# Autodesk Inventor assembly: battery
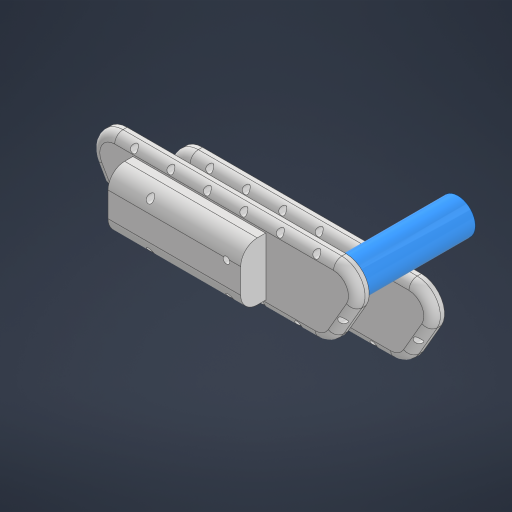
[picture p0: Inventor's stored thumbnail of the model, 512x512]
Saved by Autodesk Inventor 2024 (Build 280153000, 153)
## iProperties
Created: 2024-05-04
Part Number: battery
Document SubType Name: Assembly
Designer: markm
Author: markm
## Documents named in this file (6)
- C:\Users\markm\OneDrive\Документы\Inventor\eventide\back\battery\battery.iam
- C:\Users\markm\OneDrive\Документы\Inventor\eventide\back\battery\cell.ipt
- C:\Users\markm\OneDrive\Документы\Inventor\eventide\back\battery\frame.ipt
- C:\Users\markm\OneDrive\Документы\Inventor\eventide\back\battery\box.ipt
- C:\Users\markm\OneDrive\Документы\Inventor\eventide\back\battery\Part2.ipt
- C:\Users\markm\OneDrive\Документы\Inventor\eventide\back\battery\Part3.ipt
## Components (17 placed, 5 different names)
1. frame:1 — Mate:1, Mate:2, Flush:4, Flush:5, Mate:3, Mate:4, Mate:5
2. cell:2 — Mate:2, Flush:5
3. box:1 — Mate:3, Mate:4, Mate:5
4. Part2:1
5. Part3:1
6. cell:1 — Mate:1, Flush:4
7. cell:3
8. cell:4
9. cell:5
10. cell:6
11. cell:7
12. cell:8
13. cell:9
14. cell:10
15. cell:11
16. cell:12
17. cell:13
## Component patterns: (12 elements, first: cell:1)
## Relationships (7: Mate 5, Flush 2)
- Mate:1: frame:1 ↔ cell:1
- Mate:2: frame:1 ↔ cell:2
- Flush:4: frame:1 ↔ cell:1
- Flush:5: frame:1 ↔ cell:2
- Mate:3: frame:1 ↔ box:1
- Mate:4: frame:1 ↔ box:1
- Mate:5 (0.25 mm): frame:1 ↔ box:1
